# Autodesk Inventor assembly: one side of drive
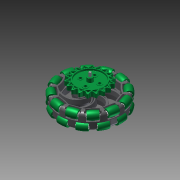
[picture p0: Inventor's stored thumbnail of the model, 180x180]
Saved by Autodesk Inventor 2014 SP1 (Build 180222100, 222)
## iProperties
Created: 2013-08-29
Part Number: one side of drive
Document SubType Name: Assembly
Designer: Ryan
Sending System: SolidWorks 2013
Last Author: Ryan
Author: Ryan
## Documents named in this file (6)
- C:\Users\Ryan\Desktop\sw\toss up 1st A bot\inventor drive\wheel assembly.iam
- C:\Users\Ryan\Desktop\sw\lib\Super Sonic Sparks VEX CAD Library\Wheels\4'' Omni-Directional Wheel.iam
- C:\Users\Ryan\Desktop\sw\lib\Aperture VEX CAD Library\Shaft\2 inch Shaft.ipt
- C:\Users\Ryan\Desktop\sw\lib\Aperture VEX CAD Library\Spacers\SPACER-0500-0125.ipt
- C:\Users\Ryan\Desktop\sw\lib\Aperture VEX CAD Library\Hardware\Shaft Collar.ipt
- C:\Users\Ryan\Desktop\sw\lib\Aperture VEX CAD Library\Sprockets\green\High Strength 18-Tooth Sprocket.ipt
## Components (5 placed, 5 different names)
1. LARGE-OMNI-WHEEL:2 [sub-assembly] — Mate:72, Mate:76
2. 2 inch shaft:1 — Flush:1, Mate:78, Mate:79
3. 18 tooth hs sprocket:1 — Mate:73, Mate:74, Mate:75, Mate:77, Mate:78, Mate:79
4. SPACER-0500-0125:1 — Flush:1, Mate:73, Mate:77
5. Shaft Collar:1 — Mate:72, Mate:74, Mate:75, Mate:76
## Relationships (9: Mate 8, Flush 1)
- Mate:72: LARGE-OMNI-WHEEL:2 ↔ Shaft Collar:1
- Flush:1 (-3.175 mm): 2 inch shaft:1 ↔ SPACER-0500-0125:1
- Mate:73: 18 tooth hs sprocket:1 ↔ SPACER-0500-0125:1
- Mate:74: 18 tooth hs sprocket:1 ↔ Shaft Collar:1
- Mate:75: 18 tooth hs sprocket:1 ↔ Shaft Collar:1
- Mate:76: LARGE-OMNI-WHEEL:2 ↔ Shaft Collar:1
- Mate:77: 18 tooth hs sprocket:1 ↔ SPACER-0500-0125:1
- Mate:78: 2 inch shaft:1 ↔ 18 tooth hs sprocket:1
- Mate:79: 2 inch shaft:1 ↔ 18 tooth hs sprocket:1
